# Autodesk Inventor assembly: Engine Assembly
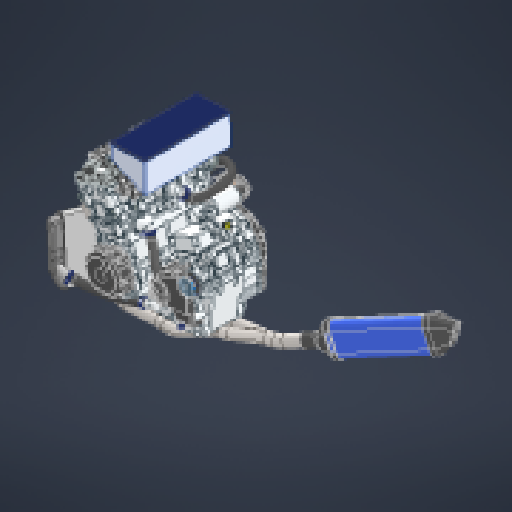
[picture p0: Inventor's stored thumbnail of the model, 512x512]
Saved by Autodesk Inventor 2027 (Build 310192000, 192)
## iProperties
Created: 2011-07-13
Part Number: Engine Assembly
Document SubType Name: Assembly
Designer: tasle
Sending System: SOLIDWORKS 2023
Last Saved Date: 2023-01-09
last saved by: Andrew
Author: tasle
## Documents named in this file (48)
- C:\Users\W Ahmad\Desktop\FSAE- Summer 2026 Project\FSAE CAD\GOGO_KART_FSAE\2005-gsxr-600-engine-model-1.snapshot.2\Engine\Engine Assembly\Engine Assembly\Engine Assembly.iam
- C:\Users\W Ahmad\Desktop\FSAE- Summer 2026 Project\FSAE CAD\GOGO_KART_FSAE\2005-gsxr-600-engine-model-1.snapshot.2\Engine\Engine Assembly\Engine Assembly\Ignition Coil.ipt
- C:\Users\W Ahmad\Desktop\FSAE- Summer 2026 Project\FSAE CAD\GOGO_KART_FSAE\2005-gsxr-600-engine-model-1.snapshot.2\Engine\Engine Assembly\Engine Assembly\Valve Cover.iam
- C:\Users\W Ahmad\Desktop\FSAE- Summer 2026 Project\FSAE CAD\GOGO_KART_FSAE\2005-gsxr-600-engine-model-1.snapshot.2\Engine\Engine Assembly\Engine Assembly\Oil Pan.ipt
- C:\Users\W Ahmad\Desktop\FSAE- Summer 2026 Project\FSAE CAD\GOGO_KART_FSAE\2005-gsxr-600-engine-model-1.snapshot.2\Engine\Engine Assembly\Engine Assembly\Oil Drain Plug.ipt
- C:\Users\W Ahmad\Desktop\FSAE- Summer 2026 Project\FSAE CAD\GOGO_KART_FSAE\2005-gsxr-600-engine-model-1.snapshot.2\Engine\Engine Assembly\Engine Assembly\Starter Gearbox Cover.ipt
- C:\Users\W Ahmad\Desktop\FSAE- Summer 2026 Project\FSAE CAD\GOGO_KART_FSAE\2005-gsxr-600-engine-model-1.snapshot.2\Engine\Engine Assembly\Engine Assembly\Suzuki_600_Oil_Inlet.ipt
- C:\Users\W Ahmad\Desktop\FSAE- Summer 2026 Project\FSAE CAD\GOGO_KART_FSAE\2005-gsxr-600-engine-model-1.snapshot.2\Engine\Engine Assembly\Engine Assembly\Engine Chain Guard.ipt
- C:\Users\W Ahmad\Desktop\FSAE- Summer 2026 Project\FSAE CAD\GOGO_KART_FSAE\2005-gsxr-600-engine-model-1.snapshot.2\Engine\Engine Assembly\Engine Assembly\Starter.ipt
- C:\Users\W Ahmad\Desktop\FSAE- Summer 2026 Project\FSAE CAD\GOGO_KART_FSAE\2005-gsxr-600-engine-model-1.snapshot.2\Engine\Engine Assembly\Engine Assembly\Cylinder Head Final.ipt
- C:\Users\W Ahmad\Desktop\FSAE- Summer 2026 Project\FSAE CAD\GOGO_KART_FSAE\2005-gsxr-600-engine-model-1.snapshot.2\Engine\Engine Assembly\Engine Assembly\Throttle Bodies.iam
- C:\Users\W Ahmad\Desktop\FSAE- Summer 2026 Project\FSAE CAD\GOGO_KART_FSAE\2005-gsxr-600-engine-model-1.snapshot.2\Engine\Engine Assembly\Engine Assembly\Exhaust Gasket.ipt
- C:\Users\W Ahmad\Desktop\FSAE- Summer 2026 Project\FSAE CAD\GOGO_KART_FSAE\2005-gsxr-600-engine-model-1.snapshot.2\Engine\Engine Assembly\Engine Assembly\2.ipt
- C:\Users\W Ahmad\Desktop\FSAE- Summer 2026 Project\FSAE CAD\GOGO_KART_FSAE\2005-gsxr-600-engine-model-1.snapshot.2\Engine\Engine Assembly\Engine Assembly\3.ipt
- C:\Users\W Ahmad\Desktop\FSAE- Summer 2026 Project\FSAE CAD\GOGO_KART_FSAE\2005-gsxr-600-engine-model-1.snapshot.2\Engine\Engine Assembly\Engine Assembly\4-2.ipt
- C:\Users\W Ahmad\Desktop\FSAE- Summer 2026 Project\FSAE CAD\GOGO_KART_FSAE\2005-gsxr-600-engine-model-1.snapshot.2\Engine\Engine Assembly\Engine Assembly\Front Collector 2-1.ipt
- C:\Users\W Ahmad\Desktop\FSAE- Summer 2026 Project\FSAE CAD\GOGO_KART_FSAE\2005-gsxr-600-engine-model-1.snapshot.2\Engine\Engine Assembly\Engine Assembly\Velocity Stack.ipt
- C:\Users\W Ahmad\Desktop\FSAE- Summer 2026 Project\FSAE CAD\GOGO_KART_FSAE\2005-gsxr-600-engine-model-1.snapshot.2\Engine\Engine Assembly\Engine Assembly\Stator Cover.ipt
- C:\Users\W Ahmad\Desktop\FSAE- Summer 2026 Project\FSAE CAD\GOGO_KART_FSAE\2005-gsxr-600-engine-model-1.snapshot.2\Engine\Engine Assembly\Engine Assembly\Head Coolant Outlet.ipt
- C:\Users\W Ahmad\Desktop\FSAE- Summer 2026 Project\FSAE CAD\GOGO_KART_FSAE\2005-gsxr-600-engine-model-1.snapshot.2\Engine\Engine Assembly\Engine Assembly\Oil Filter.ipt
- C:\Users\W Ahmad\Desktop\FSAE- Summer 2026 Project\FSAE CAD\GOGO_KART_FSAE\2005-gsxr-600-engine-model-1.snapshot.2\Engine\Engine Assembly\Engine Assembly\Oil Cooler.ipt
- C:\Users\W Ahmad\Desktop\FSAE- Summer 2026 Project\FSAE CAD\GOGO_KART_FSAE\2005-gsxr-600-engine-model-1.snapshot.2\Engine\Engine Assembly\Engine Assembly\Engine Drive Gear.ipt
- C:\Users\W Ahmad\Desktop\FSAE- Summer 2026 Project\FSAE CAD\GOGO_KART_FSAE\2005-gsxr-600-engine-model-1.snapshot.2\Engine\Engine Assembly\Engine Assembly\Block Lower.ipt
- C:\Users\W Ahmad\Desktop\FSAE- Summer 2026 Project\FSAE CAD\GOGO_KART_FSAE\2005-gsxr-600-engine-model-1.snapshot.2\Engine\Engine Assembly\Engine Assembly\Output Shaft.ipt
- C:\Users\W Ahmad\Desktop\FSAE- Summer 2026 Project\FSAE CAD\GOGO_KART_FSAE\2005-gsxr-600-engine-model-1.snapshot.2\Engine\Engine Assembly\Engine Assembly\Output Shaft Nut.ipt
- C:\Users\W Ahmad\Desktop\FSAE- Summer 2026 Project\FSAE CAD\GOGO_KART_FSAE\2005-gsxr-600-engine-model-1.snapshot.2\Engine\Engine Assembly\Engine Assembly\Starter Gearbox 2.ipt
- C:\Users\W Ahmad\Desktop\FSAE- Summer 2026 Project\FSAE CAD\GOGO_KART_FSAE\2005-gsxr-600-engine-model-1.snapshot.2\Engine\Engine Assembly\Engine Assembly\6.ipt
- C:\Users\W Ahmad\Desktop\FSAE- Summer 2026 Project\FSAE CAD\GOGO_KART_FSAE\2005-gsxr-600-engine-model-1.snapshot.2\Engine\Engine Assembly\Engine Assembly\Front Collector 2-1 Large.ipt
- C:\Users\W Ahmad\Desktop\FSAE- Summer 2026 Project\FSAE CAD\GOGO_KART_FSAE\2005-gsxr-600-engine-model-1.snapshot.2\Engine\Engine Assembly\Engine Assembly\7.ipt
- C:\Users\W Ahmad\Desktop\FSAE- Summer 2026 Project\FSAE CAD\GOGO_KART_FSAE\2005-gsxr-600-engine-model-1.snapshot.2\Engine\Engine Assembly\Engine Assembly\8.ipt
- C:\Users\W Ahmad\Desktop\FSAE- Summer 2026 Project\FSAE CAD\GOGO_KART_FSAE\2005-gsxr-600-engine-model-1.snapshot.2\Engine\Engine Assembly\Engine Assembly\9.ipt
- C:\Users\W Ahmad\Desktop\FSAE- Summer 2026 Project\FSAE CAD\GOGO_KART_FSAE\2005-gsxr-600-engine-model-1.snapshot.2\Engine\Engine Assembly\Engine Assembly\muffler.ipt
- C:\Users\W Ahmad\Desktop\FSAE- Summer 2026 Project\FSAE CAD\GOGO_KART_FSAE\2005-gsxr-600-engine-model-1.snapshot.2\Engine\Engine Assembly\Engine Assembly\Exhaust to Engine Bracket.ipt
- C:\Users\W Ahmad\Desktop\FSAE- Summer 2026 Project\FSAE CAD\GOGO_KART_FSAE\2005-gsxr-600-engine-model-1.snapshot.2\Engine\Engine Assembly\Engine Assembly\Crank Case Upper.ipt
- C:\Users\W Ahmad\Desktop\FSAE- Summer 2026 Project\FSAE CAD\GOGO_KART_FSAE\2005-gsxr-600-engine-model-1.snapshot.2\Engine\Engine Assembly\Engine Assembly\Water Pump Back Plate.ipt
- C:\Users\W Ahmad\Desktop\FSAE- Summer 2026 Project\FSAE CAD\GOGO_KART_FSAE\2005-gsxr-600-engine-model-1.snapshot.2\Engine\Engine Assembly\Engine Assembly\Water Pump.ipt
- C:\Users\W Ahmad\Desktop\FSAE- Summer 2026 Project\FSAE CAD\GOGO_KART_FSAE\2005-gsxr-600-engine-model-1.snapshot.2\Engine\Engine Assembly\Engine Assembly\Airbox.ipt
- C:\Users\W Ahmad\Desktop\FSAE- Summer 2026 Project\FSAE CAD\GOGO_KART_FSAE\2005-gsxr-600-engine-model-1.snapshot.2\Engine\Engine Assembly\Engine Assembly\Coolant Outlet Pipe.ipt
- C:\Users\W Ahmad\Desktop\FSAE- Summer 2026 Project\FSAE CAD\GOGO_KART_FSAE\2005-gsxr-600-engine-model-1.snapshot.2\Engine\Engine Assembly\Engine Assembly\Coolant Hose Clamp.ipt
- C:\Users\W Ahmad\Desktop\FSAE- Summer 2026 Project\FSAE CAD\GOGO_KART_FSAE\2005-gsxr-600-engine-model-1.snapshot.2\Engine\Engine Assembly\Engine Assembly\Coolant Inlet Pipe.ipt
- C:\Users\W Ahmad\Desktop\FSAE- Summer 2026 Project\FSAE CAD\GOGO_KART_FSAE\2005-gsxr-600-engine-model-1.snapshot.2\Engine\Engine Assembly\Engine Assembly\K&N 33-2046 - 87-95 Jeep YJ.ipt
- C:\Users\W Ahmad\Desktop\FSAE- Summer 2026 Project\FSAE CAD\GOGO_KART_FSAE\2005-gsxr-600-engine-model-1.snapshot.2\Engine\Engine Assembly\Engine Assembly\Engine Shifter Rod.ipt
- C:\Users\W Ahmad\Desktop\FSAE- Summer 2026 Project\FSAE CAD\GOGO_KART_FSAE\2005-gsxr-600-engine-model-1.snapshot.2\Engine\Engine Assembly\Engine Assembly\Cylinder Block.ipt
- C:\Users\W Ahmad\Desktop\FSAE- Summer 2026 Project\FSAE CAD\GOGO_KART_FSAE\2005-gsxr-600-engine-model-1.snapshot.2\Engine\Engine Assembly\Engine Assembly\Clutch Cover.ipt
- C:\Users\W Ahmad\Desktop\FSAE- Summer 2026 Project\FSAE CAD\GOGO_KART_FSAE\2005-gsxr-600-engine-model-1.snapshot.2\Engine\Engine Assembly\Engine Assembly\Radiator Assembly.iam
- C:\Users\W Ahmad\Desktop\FSAE- Summer 2026 Project\FSAE CAD\GOGO_KART_FSAE\2005-gsxr-600-engine-model-1.snapshot.2\Engine\Engine Assembly\Engine Assembly\Coolant Inlet Housing.ipt
- C:\Users\W Ahmad\Desktop\FSAE- Summer 2026 Project\FSAE CAD\GOGO_KART_FSAE\2005-gsxr-600-engine-model-1.snapshot.2\Engine\Engine Assembly\Engine Assembly\Pump to Head Coolant Pipe.ipt
- C:\Users\W Ahmad\Desktop\FSAE- Summer 2026 Project\FSAE CAD\GOGO_KART_FSAE\Chain-Sprocket_V1\Design Accelerator\Chain Drive1.iam
## Components (77 placed, 77 different names)
1. Ignition Coil-1
2. Ignition Coil-2
3. Ignition Coil-3
4. Ignition Coil-4
5. Valve Cover-1 [sub-assembly]
6. Oil Pan-1
7. Oil Drain Plug-1
8. Starter Gearbox Cover-1
9. Suzuki_600_Oil_Inlet-1
10. Engine Chain Guard-1
11. Starter-1
12. Cylinder Head Final-1
13. Throttle Bodies-2 [sub-assembly]
14. Exhaust Gasket-1
15. Exhaust Gasket-2
16. Exhaust Gasket-3
17. Exhaust Gasket-4
18. 2-1
19. 2-2
20. 2-3
21. 2-4
22. 3-1
23. 3-2
24. 4-2-1
25. Front Collector 2-1-1
26. Front Collector 2-1-2
27. Velocity Stack-1
28. Velocity Stack-2
29. Velocity Stack-3
30. Velocity Stack-4
31. Stator Cover-1
32. Head Coolant Outlet-1
33. Oil Filter-1
34. Oil Cooler-1
35. Engine Drive Gear-1
36. Block Lower-1
37. Output Shaft-1 — Mate:1
38. Output Shaft Nut-1
39. Starter Gearbox 2-1
40. 3-3
41. 3-4
42. 6-1
43. 6-2
44. 6-3
45. 6-4
46. 4-2-2
47. 4-2-3
48. 4-2-4
49. Front Collector 2-1 Large-1
50. 7-1
51. 8-1
52. 9-1
53. muffler-1
54. Exhaust to Engine Bracket-1
55. Exhaust to Engine Bracket-2
56. Exhaust to Engine Bracket-3
57. Exhaust to Engine Bracket-4
58. Crank Case Upper-1
59. Water Pump Back Plate-1
60. Water Pump-1
61. Airbox-1
62. Coolant Outlet Pipe-1
63. Coolant Hose Clamp-1
64. Coolant Hose Clamp-2
65. Coolant Inlet Pipe-1
66. Coolant Hose Clamp-3
67. Coolant Hose Clamp-4
68. K&N 33-2046 - 87-95 Jeep YJ-1
69. Engine Shifter Rod-2
70. Cylinder Block-1
71. Clutch Cover-3
72. Radiator Assembly-1 [sub-assembly]
73. Coolant Inlet Housing-1
74. Pump to Head Coolant Pipe-1
75. Coolant Hose Clamp-5
76. Coolant Hose Clamp-6
77. Chain Drive:1 [sub-assembly] — Mate:1
## Relationships (1: Mate 1)
- Mate:1: Output Shaft-1 ↔ Chain Drive:1
